# Autodesk Inventor assembly: 8 ball mechanism 2
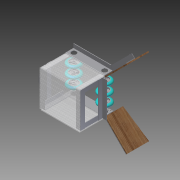
[picture p0: Inventor's stored thumbnail of the model, 180x180]
Saved by Autodesk Inventor 2012 (Build 160160000, 160)
## iProperties
Created: 2013-10-10
Part Number: 8 ball mechanism 2
Document SubType Name: Assembly
Designer: Bryce
Author: Bryce
## Documents named in this file (13)
- C:\Users\Bryce\Dropbox\Inventor Design Project Files\Independent Swerves\Inventor 2012\8 ball mechanism 2.iam
- C:\Users\Bryce\Dropbox\Inventor Design Project Files\Independent Swerves\Inventor 2012\8 ball bottom 1 by 2 L.ipt
- C:\Users\Bryce\Dropbox\Inventor Design Project Files\Independent Swerves\Inventor 2012\8 ball corner L.ipt
- C:\Users\Bryce\Dropbox\Inventor Design Project Files\Independent Swerves\Inventor 2012\8 ball corner L_MIR.ipt
- C:\Users\Bryce\Dropbox\Inventor Design Project Files\Independent Swerves\Inventor 2012\8 ball bottom 1 by 2 L_MIR.ipt
- C:\Users\Bryce\Dropbox\Inventor Design Project Files\Independent Swerves\Inventor 2012\8 ball corner L_MIR1.ipt
- C:\Users\Bryce\Dropbox\Inventor Design Project Files\Independent Swerves\Inventor 2012\8 ball corner L_MIR_MIR.ipt
- C:\Users\Bryce\Dropbox\Inventor Design Project Files\Independent Swerves\Inventor 2012\front L.ipt
- C:\Users\Bryce\Dropbox\Inventor Design Project Files\Independent Swerves\Inventor 2012\8 ball mount L.ipt
- C:\Users\Bryce\Dropbox\Inventor Design Project Files\Independent Swerves\Inventor 2012\8 ball polycarb top.ipt
- C:\Users\Bryce\Dropbox\Inventor Design Project Files\Independent Swerves\Inventor 2012\blue wheel.iam
- C:\Users\Bryce\Dropbox\Inventor Design Project Files\Independent Swerves\Inventor 2012\8 ball polycarb side.ipt
- C:\Users\Bryce\Dropbox\Inventor Design Project Files\Independent Swerves\Inventor 2012\8 ball funnel plate.ipt
## Components (21 placed, 12 different names)
1. 8 ball bottom 1 by 2 L:1 — Mate:1, Mate:2, Flush:1, Flush:2, Flush:3, Mate:10, Mate:11, Flush:11, Mate:18, Mate:21, Mate:32, Mate:34, Flush:27, Flush:28
2. 8 ball corner L:1 — Mate:1, Mate:2, Flush:1, Mate:7, Flush:8, Flush:9, Mate:14, Flush:13, Mate:15, Flush:15, Mate:23
3. 8 ball corner L_MIR:1 — Mate:6, Mate:8, Flush:10, Mate:9, Mate:10, Mate:11, Flush:11, Mate:31
4. 8 ball bottom 1 by 2 L_MIR:1 — Flush:4, Mate:3, Mate:4, Flush:5, Mate:5, Mate:12, Mate:13, Flush:12, Mate:17, Mate:20, Mate:30, Flush:22, Mate:35, Flush:26
5. 8 ball corner L_MIR1:1 — Flush:4, Mate:3, Mate:4
6. 8 ball corner L_MIR_MIR:1 — Flush:6, Flush:7, Mate:12, Mate:13, Flush:12, Mate:26, Mate:29
7. front L:1 — Mate:6, Flush:6, Flush:7
8. 8 ball mount L:1 — Mate:7, Flush:8, Flush:9
9. front L:2 — Mate:8, Flush:10, Mate:9, Mate:16, Flush:20
10. front L:3 — Mate:14, Flush:13, Mate:15, Flush:14
11. 8 ball polycarb top:1 — Mate:16, Flush:14, Flush:15, Flush:21
12. blue wheel:1 [sub-assembly] — Mate:20, Mate:22, Flush:17, Mate:26, Mate:27
13. blue wheel:2 [sub-assembly] — Mate:21, Flush:16, Mate:28
14. blue wheel:3 [sub-assembly] — Mate:22, Flush:16, Flush:17, Mate:27, Mate:28
15. blue wheel:4 [sub-assembly] — Mate:19, Flush:18, Flush:19, Mate:24, Mate:25
16. blue wheel:5 [sub-assembly] — Mate:18, Flush:19, Mate:23, Mate:24
17. blue wheel:6 [sub-assembly] — Mate:17, Mate:19, Flush:18, Mate:25
18. 8 ball polycarb side:1 — Mate:29, Mate:30, Flush:20
19. 8 ball polycarb side:2 — Mate:31, Mate:32, Flush:21
20. 8 ball funnel plate:1 — Flush:22, Mate:35, Flush:26
21. 8 ball funnel plate:2 — Mate:34, Flush:27, Flush:28
## Relationships (59: Mate 34, Flush 25)
- Mate:1: 8 ball bottom 1 by 2 L:1 ↔ 8 ball corner L:1
- Mate:2: 8 ball bottom 1 by 2 L:1 ↔ 8 ball corner L:1
- Flush:1: 8 ball bottom 1 by 2 L:1 ↔ 8 ball corner L:1
- Flush:2 (-114.3 mm): 8 ball bottom 1 by 2 L:1
- Flush:3 (101.6 mm): 8 ball bottom 1 by 2 L:1
- Flush:4: 8 ball bottom 1 by 2 L_MIR:1 ↔ 8 ball corner L_MIR1:1
- Mate:3: 8 ball bottom 1 by 2 L_MIR:1 ↔ 8 ball corner L_MIR1:1
- Mate:4: 8 ball bottom 1 by 2 L_MIR:1 ↔ 8 ball corner L_MIR1:1
- Flush:5 (-114.3 mm): 8 ball bottom 1 by 2 L_MIR:1
- Mate:5 (101.6 mm): 8 ball bottom 1 by 2 L_MIR:1
- Mate:6: 8 ball corner L_MIR:1 ↔ front L:1
- Flush:6: 8 ball corner L_MIR_MIR:1 ↔ front L:1
- Flush:7: 8 ball corner L_MIR_MIR:1 ↔ front L:1
- Mate:7: 8 ball corner L:1 ↔ 8 ball mount L:1
- Flush:8: 8 ball corner L:1 ↔ 8 ball mount L:1
- Flush:9 (34.925 mm): 8 ball corner L:1 ↔ 8 ball mount L:1
- Mate:8: 8 ball corner L_MIR:1 ↔ front L:2
- Flush:10: 8 ball corner L_MIR:1 ↔ front L:2
- Mate:9: 8 ball corner L_MIR:1 ↔ front L:2
- Mate:10: 8 ball bottom 1 by 2 L:1 ↔ 8 ball corner L_MIR:1
- Mate:11: 8 ball bottom 1 by 2 L:1 ↔ 8 ball corner L_MIR:1
- Flush:11: 8 ball bottom 1 by 2 L:1 ↔ 8 ball corner L_MIR:1
- Mate:12: 8 ball bottom 1 by 2 L_MIR:1 ↔ 8 ball corner L_MIR_MIR:1
- Mate:13: 8 ball bottom 1 by 2 L_MIR:1 ↔ 8 ball corner L_MIR_MIR:1
- Flush:12: 8 ball bottom 1 by 2 L_MIR:1 ↔ 8 ball corner L_MIR_MIR:1
- Mate:14: 8 ball corner L:1 ↔ front L:3
- Flush:13: 8 ball corner L:1 ↔ front L:3
- Mate:15: 8 ball corner L:1 ↔ front L:3
- Mate:16: front L:2 ↔ 8 ball polycarb top:1
- Flush:14: front L:3 ↔ 8 ball polycarb top:1
- Flush:15 (-0.254 mm): 8 ball corner L:1 ↔ 8 ball polycarb top:1
- Mate:17: 8 ball bottom 1 by 2 L_MIR:1 ↔ blue wheel:6
- Mate:18: 8 ball bottom 1 by 2 L:1 ↔ blue wheel:5
- Mate:19: blue wheel:4 ↔ blue wheel:6
- Mate:20: 8 ball bottom 1 by 2 L_MIR:1 ↔ blue wheel:1
- Mate:21: 8 ball bottom 1 by 2 L:1 ↔ blue wheel:2
- Mate:22: blue wheel:1 ↔ blue wheel:3
- Flush:16: blue wheel:2 ↔ blue wheel:3
- Flush:17: blue wheel:1 ↔ blue wheel:3
- Flush:18: blue wheel:4 ↔ blue wheel:6
- Flush:19: blue wheel:4 ↔ blue wheel:5
- Mate:23 (37.3062 mm): 8 ball corner L:1 ↔ blue wheel:5
- Mate:24 (37.3062 mm): blue wheel:4 ↔ blue wheel:5
- Mate:25 (37.3062 mm): blue wheel:4 ↔ blue wheel:6
- Mate:26 (37.3062 mm): 8 ball corner L_MIR_MIR:1 ↔ blue wheel:1
- Mate:27 (37.3062 mm): blue wheel:1 ↔ blue wheel:3
- Mate:28 (37.3062 mm): blue wheel:2 ↔ blue wheel:3
- Mate:29: 8 ball corner L_MIR_MIR:1 ↔ 8 ball polycarb side:1
- Mate:30: 8 ball bottom 1 by 2 L_MIR:1 ↔ 8 ball polycarb side:1
- Flush:20: front L:2 ↔ 8 ball polycarb side:1
- Mate:31: 8 ball corner L_MIR:1 ↔ 8 ball polycarb side:2
- Mate:32: 8 ball bottom 1 by 2 L:1 ↔ 8 ball polycarb side:2
- Flush:21: 8 ball polycarb top:1 ↔ 8 ball polycarb side:2
- Flush:22: 8 ball bottom 1 by 2 L_MIR:1 ↔ 8 ball funnel plate:1
- Mate:34: 8 ball bottom 1 by 2 L:1 ↔ 8 ball funnel plate:2
- Mate:35: 8 ball bottom 1 by 2 L_MIR:1 ↔ 8 ball funnel plate:1
- Flush:26: 8 ball bottom 1 by 2 L_MIR:1 ↔ 8 ball funnel plate:1
- Flush:27: 8 ball bottom 1 by 2 L:1 ↔ 8 ball funnel plate:2
- Flush:28: 8 ball bottom 1 by 2 L:1 ↔ 8 ball funnel plate:2
